# Autodesk Inventor assembly: FCFM-CNAF-3
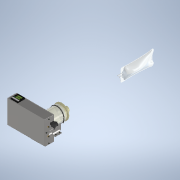
[picture p0: Inventor's stored thumbnail of the model, 180x180]
Saved by Autodesk Inventor 2020.3 (Build 243373000, 373)
## iProperties
Created: 2020-06-30
Part Number: FCFM-CNAF-3
Document SubType Name: Assembly
Designer: Bruno
Author: Bruno
## Documents named in this file (27)
- C:\Users\Bruno\Desktop\CNAF\CNAF-3\FCFM-CNAF-3.iam
- C:\Users\Bruno\Desktop\CNAF\CNAF-3\base_v7.ipt
- C:\Users\Bruno\Desktop\CNAF\CNAF-3\tapa_v7.ipt
- C:\Users\Bruno\Desktop\CNAF\CNAF-3\Tuerca Remachable M4.ipt
- C:\Users\Bruno\Desktop\CNAF\CNAF-3\Perno Parker DIN912 M4x0.7x10-8.8.ipt
- C:\Users\Bruno\Desktop\CNAF\CNAF-3\Temp Controlador RexC100.ipt
- C:\Users\Bruno\Desktop\CNAF\CNAF-3\Perno Parker DIN912 M4x0.7x40-8.8.ipt
- C:\Users\Bruno\Desktop\CNAF\CNAF-3\Sello Plato Oring 2-343.ipt
- C:\Users\Bruno\Desktop\CNAF\CNAF-3\Plato Calefactor.ipt
- C:\Users\Bruno\Desktop\CNAF\CNAF-3\Barra fijación calefactor V2.ipt
- C:\Users\Bruno\Desktop\CNAF\CNAF-3\Tuerca DIN934-M4.ipt
- C:\Users\Bruno\Desktop\CNAF\CNAF-3\Termocupla.ipt
- C:\Users\Bruno\Desktop\CNAF\CNAF-3\Calefactor630W.ipt
- C:\Users\Bruno\Desktop\CNAF\CNAF-3\Solid State Rele SSR40DA.ipt
- C:\Users\Bruno\Desktop\CNAF\CNAF-3\Vaso precipitado 600ml-De90-Di84-H120.ipt
- C:\Users\Bruno\Desktop\CNAF\CNAF-3\Sujetador Vaso.ipt
- C:\Users\Bruno\Desktop\CNAF\CNAF-3\Sujetador Porta Suero.iam
- C:\Users\Bruno\Desktop\CNAF\CNAF-3\Switch OnOff 240V20A.ipt
- C:\Users\Bruno\Desktop\CNAF\CNAF-3\Conector IEC C14 Macho Panel.ipt
- C:\Users\Bruno\Desktop\CNAF\CNAF-3\Tapa V2.iam
- C:\Users\Bruno\Desktop\CNAF\CNAF-3\Oring 2-159 SujetaVaso.ipt
- C:\Users\Bruno\Desktop\CNAF\CNAF-3\Bolsa Agua Destilada.ipt
- C:\Users\Bruno\Desktop\CNAF\CNAF-3\Arandela Presion DIN127B D4.ipt
- C:\Users\Bruno\Desktop\CNAF\CNAF-3\Prisionero DIN913-M5x5.ipt
- C:\Users\Bruno\Desktop\CNAF\CNAF-3\Perilla 1-4UNC Star Knob.ipt
- C:\Users\Bruno\Desktop\CNAF\CNAF-3\Perno Parker Avellanado DIN7991 M3x0.5x10-8.8.ipt
- C:\Users\Bruno\Desktop\CNAF\CNAF-3\Tuerca DIN934-M3.ipt
## Components (67 placed, 26 different names)
1. base_v7:1 — Mate:1, Flush:1, Flush:2, Cylindrical:1, Cylindrical:2, Cylindrical:3, Cylindrical:4, Cylindrical:5, Cylindrical:6, Cylindrical:7, Cylindrical:8, Cylindrical:9, Cylindrical:10, Mate:2, Mate:3, Mate:4, Mate:5, Mate:6, Mate:7, Cylindrical:28, Cylindrical:29, Mate:8, Mate:9, Mate:10, Cylindrical:43, Cylindrical:69, Cylindrical:70
2. tapa_v7:1 — Mate:1, Flush:1, Flush:2, Cylindrical:11, Cylindrical:12, Cylindrical:13, Cylindrical:14, Cylindrical:15, Cylindrical:16, Cylindrical:17, Cylindrical:18, Cylindrical:19, Cylindrical:20, Rotational:1, Rotational:2, Cylindrical:21, Cylindrical:33, Cylindrical:34, Cylindrical:35, Cylindrical:36
3. Tuerca Remachable M4:1 — Cylindrical:1
4. Tuerca Remachable M4:2 — Cylindrical:4
5. Tuerca Remachable M4:3 — Cylindrical:2
6. Tuerca Remachable M4:4 — Cylindrical:3
7. Tuerca Remachable M4:5 — Cylindrical:7
8. Tuerca Remachable M4:6 — Cylindrical:6
9. Tuerca Remachable M4:7 — Cylindrical:5
10. Tuerca Remachable M4:8 — Cylindrical:10
11. Tuerca Remachable M4:9 — Cylindrical:9
12. Tuerca Remachable M4:10 — Cylindrical:8
13. Perno Parker DIN912 M4x0.7x10-8.8:1 — Cylindrical:11
14. Perno Parker DIN912 M4x0.7x10-8.8:2 — Cylindrical:13
15. Perno Parker DIN912 M4x0.7x10-8.8:3 — Cylindrical:12
16. Perno Parker DIN912 M4x0.7x10-8.8:4 — Cylindrical:14
17. Perno Parker DIN912 M4x0.7x10-8.8:5 — Cylindrical:15
18. Perno Parker DIN912 M4x0.7x10-8.8:6 — Cylindrical:16
19. Perno Parker DIN912 M4x0.7x10-8.8:7 — Cylindrical:17
20. Perno Parker DIN912 M4x0.7x10-8.8:8 — Cylindrical:20
21. Perno Parker DIN912 M4x0.7x10-8.8:9 — Cylindrical:19
22. Perno Parker DIN912 M4x0.7x10-8.8:10 — Cylindrical:18
23. Temp Controlador RexC100:1 — Mate:2, Mate:3, Mate:4
24. Perno Parker DIN912 M4x0.7x40-8.8:1 — Rotational:1
25. Perno Parker DIN912 M4x0.7x40-8.8:2 — Rotational:2, Insert:1
26. Sello Plato Oring 2-343:1 — Cylindrical:21, Cylindrical:22
27. Plato Calefactor:1 — Cylindrical:22, Cylindrical:25, Cylindrical:26, Cylindrical:27, Cylindrical:58, Cylindrical:59
28. Barra fijación calefactor V2:1 — Insert:1, Cylindrical:23, Cylindrical:24
29. Tuerca DIN934-M4:1 — Cylindrical:23
30. Tuerca DIN934-M4:2 — Cylindrical:24
31. Termocupla:1 — Cylindrical:25
32. Calefactor630W:1 — Cylindrical:26
33. SSR-XXDA:1 — Mate:5, Mate:6, Mate:7
34. Vaso precipitado 600ml-De90-Di84-H120:1 — Cylindrical:27, Cylindrical:44, Cylindrical:48
35. Tuerca Remachable M4:11 — Cylindrical:28
36. Tuerca Remachable M4:12 — Cylindrical:29, Cylindrical:49
37. Perno Parker DIN912 M4x0.7x10-8.8:11 — Cylindrical:51
38. Perno Parker DIN912 M4x0.7x10-8.8:12 — Cylindrical:50
39. Tuerca Remachable M4:13 — Cylindrical:33
40. Tuerca Remachable M4:14 — Cylindrical:34, Cylindrical:37
41. Tuerca Remachable M4:15 — Cylindrical:35, Cylindrical:38
42. Tuerca Remachable M4:16 — Cylindrical:36
43. Sujetador Porta Suero:1 [sub-assembly] — Cylindrical:37, Cylindrical:39, Cylindrical:40, Cylindrical:52, Cylindrical:53, Cylindrical:66
44. Sujetador Porta Suero:2 [sub-assembly] — Cylindrical:38, Cylindrical:41, Cylindrical:42, Cylindrical:54, Cylindrical:55
45. Perno Parker DIN912 M4x0.7x10-8.8:13 — Cylindrical:39
46. Perno Parker DIN912 M4x0.7x10-8.8:14 — Cylindrical:40
47. Perno Parker DIN912 M4x0.7x10-8.8:15 — Cylindrical:42
48. Perno Parker DIN912 M4x0.7x10-8.8:16 — Cylindrical:41
49. Switch OnOff 240V20A:1 — Mate:8, Mate:9, Mate:10
50. Conector IEC C14 Macho Panel:1 — Cylindrical:43, Cylindrical:67, Cylindrical:68
51. Tapa V2:1 [sub-assembly] — Cylindrical:44
52. Oring 2-159 SujetaVaso:1 — Cylindrical:48
53. Sujetador Vaso:1 — Cylindrical:49, Cylindrical:50, Cylindrical:51
54. Bolsa Agua Destilada:1
55. Arandela Presion DIN127B D4:1 — Cylindrical:52, Cylindrical:57
56. Arandela Presion DIN127B D4:2 — Cylindrical:53, Cylindrical:56
57. Tuerca DIN934-M4:3 — Cylindrical:54
58. Tuerca DIN934-M4:4 — Cylindrical:55
59. Perno Parker DIN912 M4x0.7x10-8.8:17 — Cylindrical:57
60. Perno Parker DIN912 M4x0.7x10-8.8:18 — Cylindrical:56
61. Prisionero DIN913-M5x5:1 — Cylindrical:59
62. Prisionero DIN913-M5x5:2 — Cylindrical:58
63. Perilla 1-4UNC Star Knob:1 — Cylindrical:66
64. Perno Parker Avellanado DIN7991 M3x0.5x10-8.8:1 — Cylindrical:67
65. Perno Parker Avellanado DIN7991 M3x0.5x10-8.8:2 — Cylindrical:68
66. Tuerca DIN934-M3:1 — Cylindrical:69
67. Tuerca DIN934-M3:2 — Cylindrical:70
## Relationships (73: CylindricalJoint 58, Mate 10, Flush 2, RevoluteJoint 2, Insert 1)
- Mate:1 (1 mm): base_v7:1 ↔ tapa_v7:1
- Flush:1 (1 mm): base_v7:1 ↔ tapa_v7:1
- Flush:2: base_v7:1 ↔ tapa_v7:1
- Cylindrical:1: base_v7:1 ↔ Tuerca Remachable M4:1
- Cylindrical:2: base_v7:1 ↔ Tuerca Remachable M4:3
- Cylindrical:3: base_v7:1 ↔ Tuerca Remachable M4:4
- Cylindrical:4: base_v7:1 ↔ Tuerca Remachable M4:2
- Cylindrical:5: base_v7:1 ↔ Tuerca Remachable M4:7
- Cylindrical:6: base_v7:1 ↔ Tuerca Remachable M4:6
- Cylindrical:7: base_v7:1 ↔ Tuerca Remachable M4:5
- Cylindrical:8: base_v7:1 ↔ Tuerca Remachable M4:10
- Cylindrical:9: base_v7:1 ↔ Tuerca Remachable M4:9
- Cylindrical:10: base_v7:1 ↔ Tuerca Remachable M4:8
- Cylindrical:11: tapa_v7:1 ↔ Perno Parker DIN912 M4x0.7x10-8.8:1
- Cylindrical:12: tapa_v7:1 ↔ Perno Parker DIN912 M4x0.7x10-8.8:3
- Cylindrical:13: tapa_v7:1 ↔ Perno Parker DIN912 M4x0.7x10-8.8:2
- Cylindrical:14: tapa_v7:1 ↔ Perno Parker DIN912 M4x0.7x10-8.8:4
- Cylindrical:15: tapa_v7:1 ↔ Perno Parker DIN912 M4x0.7x10-8.8:5
- Cylindrical:16: tapa_v7:1 ↔ Perno Parker DIN912 M4x0.7x10-8.8:6
- Cylindrical:17: tapa_v7:1 ↔ Perno Parker DIN912 M4x0.7x10-8.8:7
- Cylindrical:18: tapa_v7:1 ↔ Perno Parker DIN912 M4x0.7x10-8.8:10
- Cylindrical:19: tapa_v7:1 ↔ Perno Parker DIN912 M4x0.7x10-8.8:9
- Cylindrical:20: tapa_v7:1 ↔ Perno Parker DIN912 M4x0.7x10-8.8:8
- Mate:2: base_v7:1 ↔ Temp Controlador RexC100:1
- Mate:3: base_v7:1 ↔ Temp Controlador RexC100:1
- Mate:4: base_v7:1 ↔ Temp Controlador RexC100:1
- Rotational:1 [RevoluteJoint]: tapa_v7:1 ↔ Perno Parker DIN912 M4x0.7x40-8.8:1
- Rotational:2 [RevoluteJoint]: tapa_v7:1 ↔ Perno Parker DIN912 M4x0.7x40-8.8:2
- Cylindrical:21: tapa_v7:1 ↔ Sello Plato Oring 2-343:1
- Cylindrical:22: Sello Plato Oring 2-343:1 ↔ Plato Calefactor:1
- Insert:1 (10.67 mm): Perno Parker DIN912 M4x0.7x40-8.8:2 ↔ Barra fijación calefactor V2:1
- Cylindrical:23: Barra fijación calefactor V2:1 ↔ Tuerca DIN934-M4:1
- Cylindrical:24: Barra fijación calefactor V2:1 ↔ Tuerca DIN934-M4:2
- Cylindrical:25: Plato Calefactor:1 ↔ Termocupla:1
- Cylindrical:26: Plato Calefactor:1 ↔ Calefactor630W:1
- Mate:5: base_v7:1 ↔ SSR-XXDA:1
- Mate:6 (3 mm): base_v7:1 ↔ SSR-XXDA:1
- Mate:7 (15 mm): base_v7:1 ↔ SSR-XXDA:1
- Cylindrical:27: Plato Calefactor:1 ↔ Vaso precipitado 600ml-De90-Di84-H120:1
- Cylindrical:28: base_v7:1 ↔ Tuerca Remachable M4:11
- Cylindrical:29: base_v7:1 ↔ Tuerca Remachable M4:12
- Cylindrical:33: tapa_v7:1 ↔ Tuerca Remachable M4:13
- Cylindrical:34: tapa_v7:1 ↔ Tuerca Remachable M4:14
- Cylindrical:35: tapa_v7:1 ↔ Tuerca Remachable M4:15
- Cylindrical:36: tapa_v7:1 ↔ Tuerca Remachable M4:16
- Cylindrical:37: Tuerca Remachable M4:14 ↔ Sujetador Porta Suero:1
- Cylindrical:38: Tuerca Remachable M4:15 ↔ Sujetador Porta Suero:2
- Cylindrical:39: Sujetador Porta Suero:1 ↔ Perno Parker DIN912 M4x0.7x10-8.8:13
- Cylindrical:40: Sujetador Porta Suero:1 ↔ Perno Parker DIN912 M4x0.7x10-8.8:14
- Cylindrical:41: Sujetador Porta Suero:2 ↔ Perno Parker DIN912 M4x0.7x10-8.8:16
- Cylindrical:42: Sujetador Porta Suero:2 ↔ Perno Parker DIN912 M4x0.7x10-8.8:15
- Mate:8: base_v7:1 ↔ Switch OnOff 240V20A:1
- Mate:9: base_v7:1 ↔ Switch OnOff 240V20A:1
- Mate:10: base_v7:1 ↔ Switch OnOff 240V20A:1
- Cylindrical:43: base_v7:1 ↔ Conector IEC C14 Macho Panel:1
- Cylindrical:44: Vaso precipitado 600ml-De90-Di84-H120:1 ↔ Tapa V2:1
- Cylindrical:48: Vaso precipitado 600ml-De90-Di84-H120:1 ↔ Oring 2-159 SujetaVaso:1
- Cylindrical:49: Tuerca Remachable M4:12 ↔ Sujetador Vaso:1
- Cylindrical:50: Perno Parker DIN912 M4x0.7x10-8.8:12 ↔ Sujetador Vaso:1
- Cylindrical:51: Perno Parker DIN912 M4x0.7x10-8.8:11 ↔ Sujetador Vaso:1
- Cylindrical:52: Sujetador Porta Suero:1 ↔ Arandela Presion DIN127B D4:1
- Cylindrical:53: Sujetador Porta Suero:1 ↔ Arandela Presion DIN127B D4:2
- Cylindrical:54: Sujetador Porta Suero:2 ↔ Tuerca DIN934-M4:3
- Cylindrical:55: Sujetador Porta Suero:2 ↔ Tuerca DIN934-M4:4
- Cylindrical:56: Arandela Presion DIN127B D4:2 ↔ Perno Parker DIN912 M4x0.7x10-8.8:18
- Cylindrical:57: Arandela Presion DIN127B D4:1 ↔ Perno Parker DIN912 M4x0.7x10-8.8:17
- Cylindrical:58: Plato Calefactor:1 ↔ Prisionero DIN913-M5x5:2
- Cylindrical:59: Plato Calefactor:1 ↔ Prisionero DIN913-M5x5:1
- Cylindrical:66: Sujetador Porta Suero:1 ↔ Perilla 1-4UNC Star Knob:1
- Cylindrical:67: Conector IEC C14 Macho Panel:1 ↔ Perno Parker Avellanado DIN7991 M3x0.5x10-8.8:1
- Cylindrical:68: Conector IEC C14 Macho Panel:1 ↔ Perno Parker Avellanado DIN7991 M3x0.5x10-8.8:2
- Cylindrical:69: base_v7:1 ↔ Tuerca DIN934-M3:1
- Cylindrical:70: base_v7:1 ↔ Tuerca DIN934-M3:2
